# Autodesk Inventor assembly: GPS-Compass_assembly
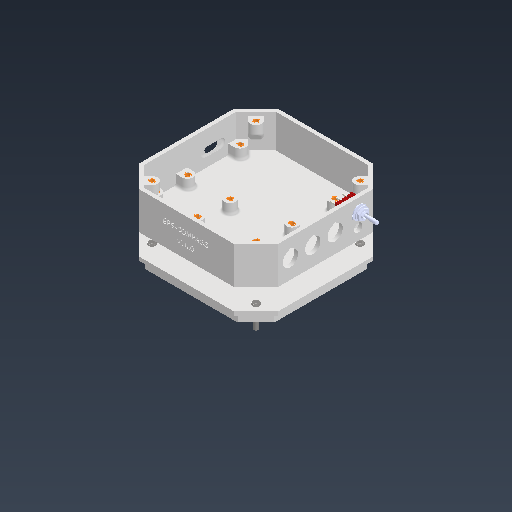
[picture p0: Inventor's stored thumbnail of the model, 512x512]
Saved by Autodesk Inventor 2026.2 (Build 302298000, 298)
## iProperties
Created: 2025-11-19
Part Number: GPS-Compass_assembly
Document SubType Name: Assembly
Designer: MenMe
Author: MenMe
## Documents named in this file (7)
- C:\Users\MenMe\GitHub\GPS-Compass\Mechanical\GPS-Compass_assembly\GPS-Compass_assembly.iam
- C:\Users\MenMe\GitHub\GPS-Compass\Mechanical\GPS-Compass_assembly\GPS-Compass_box.ipt
- C:\Users\MenMe\GitHub\GPS-Compass\Mechanical\GPS-Compass_assembly\GPS-Compass_top.ipt
- C:\Users\MenMe\GitHub\GPS-Compass\Mechanical\GPS-Compass_assembly\GPS-Compass_plexi.ipt
- C:\Users\MenMe\GitHub\GPS-Compass\Mechanical\GPS-Compass_assembly\DODGE INSERT M3X4(D5-Dill4.8)\DODGE INSERT M3X4(D5-Dill4.8)\DODGE INSERT M3X4(D5-Dill4.8).ipt
- C:\Users\MenMe\Documents\Inventor\Content Center Files\R2026\en-US\ISO 4762(2)\ISO 4762 - M3 x 16ISO.ipt
- C:\Users\MenMe\GitHub\GPS-Compass\Mechanical\GPS-Compass_assembly\parts\Toggle_Switch_SPDT_PCB\Toggle_Switch_SPDT_PCB\Toggle_Switch_SPDT_PCB.iam
## Components (21 placed, 6 different names)
1. GPS-Compass_box:1 — Mate:2, Mate:3, Mate:4, Insert:1, Insert:7, Insert:8, Insert:9, Mate:11, Insert:10, Insert:11, Insert:12, Insert:13, Insert:14, Insert:15
2. GPS-Compass_top:1 — Mate:2, Mate:3, Mate:4, Mate:8, Mate:9, Mate:10, Insert:2, Insert:3, Insert:4, Insert:5
3. GPS-Compass_plexi:1 — Mate:8, Mate:9, Mate:10
4. DODGE INSERT M3X4(D5-Dill4.8):1 — Insert:1
5. ISO 4762 M3 x 16:1 — Insert:2
6. ISO 4762 M3 x 16:2 — Insert:3
7. ISO 4762 M3 x 16:3 — Insert:4
8. ISO 4762 M3 x 16:4 — Insert:5
9. DODGE INSERT M3X4(D5-Dill4.8):3 — Insert:7
10. DODGE INSERT M3X4(D5-Dill4.8):4 — Insert:8
11. DODGE INSERT M3X4(D5-Dill4.8):5 — Insert:9
12. DODGE INSERT M3X4(D5-Dill4.8):6 — Mate:11
13. DODGE INSERT M3X4(D5-Dill4.8):7 — Insert:10
14. DODGE INSERT M3X4(D5-Dill4.8):8 — Insert:11
15. DODGE INSERT M3X4(D5-Dill4.8):9 — Insert:12
16. DODGE INSERT M3X4(D5-Dill4.8):10 — Insert:13
17. DODGE INSERT M3X4(D5-Dill4.8):11 — Insert:14
18. DODGE INSERT M3X4(D5-Dill4.8):12 — Insert:15
19. DODGE INSERT M3X4(D5-Dill4.8):13
20. DODGE INSERT M3X4(D5-Dill4.8):14
21. Toggle_Switch_SPDT_PCB:1 [sub-assembly]
## Relationships (21: Insert 14, Mate 7)
- Mate:2 (-50 mm): GPS-Compass_box:1 ↔ GPS-Compass_top:1
- Mate:3: GPS-Compass_box:1 ↔ GPS-Compass_top:1
- Mate:4: GPS-Compass_box:1 ↔ GPS-Compass_top:1
- Mate:8: GPS-Compass_top:1 ↔ GPS-Compass_plexi:1
- Mate:9: GPS-Compass_top:1 ↔ GPS-Compass_plexi:1
- Mate:10: GPS-Compass_top:1 ↔ GPS-Compass_plexi:1
- Insert:1: GPS-Compass_box:1 ↔ DODGE INSERT M3X4(D5-Dill4.8):1
- Insert:2: GPS-Compass_top:1 ↔ ISO 4762 M3 x 16:1
- Insert:3: GPS-Compass_top:1 ↔ ISO 4762 M3 x 16:2
- Insert:4: GPS-Compass_top:1 ↔ ISO 4762 M3 x 16:3
- Insert:5: GPS-Compass_top:1 ↔ ISO 4762 M3 x 16:4
- Insert:7: GPS-Compass_box:1 ↔ DODGE INSERT M3X4(D5-Dill4.8):3
- Insert:8: GPS-Compass_box:1 ↔ DODGE INSERT M3X4(D5-Dill4.8):4
- Insert:9: GPS-Compass_box:1 ↔ DODGE INSERT M3X4(D5-Dill4.8):5
- Mate:11: GPS-Compass_box:1 ↔ DODGE INSERT M3X4(D5-Dill4.8):6
- Insert:10: GPS-Compass_box:1 ↔ DODGE INSERT M3X4(D5-Dill4.8):7
- Insert:11: GPS-Compass_box:1 ↔ DODGE INSERT M3X4(D5-Dill4.8):8
- Insert:12: GPS-Compass_box:1 ↔ DODGE INSERT M3X4(D5-Dill4.8):9
- Insert:13: GPS-Compass_box:1 ↔ DODGE INSERT M3X4(D5-Dill4.8):10
- Insert:14: GPS-Compass_box:1 ↔ DODGE INSERT M3X4(D5-Dill4.8):11
- Insert:15: GPS-Compass_box:1 ↔ DODGE INSERT M3X4(D5-Dill4.8):12
